# Autodesk Inventor assembly: robot
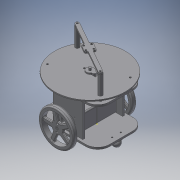
[picture p0: Inventor's stored thumbnail of the model, 180x180]
Saved by Autodesk Inventor 2017 (Build 210142000, 142)
## iProperties
Created: 2017-06-15
Part Number: robot
Document SubType Name: Assembly
Designer: millerid
Author: millerid
## Documents named in this file (13)
- U:\Research\Swarms\RobotModel\robot.iam
- U:\Research\Swarms\RobotModel\pcb.ipt
- U:\Research\Swarms\RobotModel\SG92R.ipt
- U:\Research\Swarms\RobotModel\NEMA11.ipt
- U:\Research\Swarms\RobotModel\halfincaster.ipt
- U:\Research\Swarms\RobotModel\1_5V_holder4AA.iam
- U:\Research\Swarms\RobotModel\Pololu 60mm Wheel.ipt
- U:\Research\Swarms\RobotModel\base_plate.ipt
- U:\Research\Swarms\RobotModel\side_plate.ipt
- U:\Research\Swarms\RobotModel\top_plate.ipt
- U:\Research\Swarms\RobotModel\quarterin_spacer.ipt
- U:\Research\Swarms\RobotModel\led_brace.ipt
- U:\Research\Swarms\RobotModel\oneandquarterstandoff.ipt
## Components (20 placed, 12 different names)
1. pcb:1 — Mate:46, Mate:47, Mate:48, Mate:64, Mate:65, Mate:67, Mate:70, Mate:71, Mate:72, Mate:73, Mate:74
2. SG92R:1 — Mate:46, Mate:47, Mate:70
3. NEMA11:1 — Mate:3, Mate:19
4. NEMA11:2 — Mate:14, Mate:15, Mate:20, Mate:61
5. halfincaster:1 — Mate:56, Mate:57
6. 1_5V_holder4AA:1 [sub-assembly] — Mate:60, Mate:61
7. Pololu 60mm Wheel:1 — Mate:3
8. halfincaster:2 — Mate:54, Mate:55, Mate:75
9. base_plate:1 — Mate:51, Mate:52, Mate:53, Mate:54, Mate:55, Mate:56, Mate:57, Mate:58, Mate:59, Mate:60, Mate:75
10. side_plate:1 — Mate:14, Mate:15, Mate:22, Mate:23, Mate:58, Mate:59
11. side_plate:2 — Mate:19
12. Pololu 60mm Wheel:2 — Mate:20
13. top_plate:1 — Mate:22, Mate:23, Mate:62, Mate:63, Mate:66, Mate:68, Mate:69
14. led_brace:1 — Mate:36, Mate:37, Mate:38, Mate:40
15. oneandquarterstandoff:1 — Mate:36, Mate:37, Mate:74
16. oneandquarterstandoff:2 — Mate:38, Mate:40, Mate:48, Mate:73
17. quarterin_spacer:1 — Mate:62, Mate:63, Mate:64, Mate:65
18. quarterin_spacer:2 — Mate:69, Mate:72
19. quarterin_spacer:3 — Mate:66, Mate:67
20. quarterin_spacer:4 — Mate:68, Mate:71
## Relationships (39: Mate 39)
- Mate:3: NEMA11:1 ↔ Pololu 60mm Wheel:1
- Mate:14: NEMA11:2 ↔ side_plate:1
- Mate:15: NEMA11:2 ↔ side_plate:1
- Mate:19: NEMA11:1 ↔ side_plate:2
- Mate:20: NEMA11:2 ↔ Pololu 60mm Wheel:2
- Mate:22: side_plate:1 ↔ top_plate:1
- Mate:23: side_plate:1 ↔ top_plate:1
- Mate:36: led_brace:1 ↔ oneandquarterstandoff:1
- Mate:37: led_brace:1 ↔ oneandquarterstandoff:1
- Mate:38 (0.1 mm): led_brace:1 ↔ oneandquarterstandoff:2
- Mate:40: led_brace:1 ↔ oneandquarterstandoff:2
- Mate:46: pcb:1 ↔ SG92R:1
- Mate:47: pcb:1 ↔ SG92R:1
- Mate:48: pcb:1 ↔ oneandquarterstandoff:2
- Mate:51: base_plate:1
- Mate:52: base_plate:1
- Mate:53: base_plate:1
- Mate:54: halfincaster:2 ↔ base_plate:1
- Mate:55: halfincaster:2 ↔ base_plate:1
- Mate:56: halfincaster:1 ↔ base_plate:1
- Mate:57: halfincaster:1 ↔ base_plate:1
- Mate:58: base_plate:1 ↔ side_plate:1
- Mate:59: base_plate:1 ↔ side_plate:1
- Mate:60: 1_5V_holder4AA:1 ↔ base_plate:1
- Mate:61: NEMA11:2 ↔ 1_5V_holder4AA:1
- Mate:62: top_plate:1 ↔ quarterin_spacer:1
- Mate:63: top_plate:1 ↔ quarterin_spacer:1
- Mate:64: pcb:1 ↔ quarterin_spacer:1
- Mate:65: pcb:1 ↔ quarterin_spacer:1
- Mate:66: top_plate:1 ↔ quarterin_spacer:3
- Mate:67: pcb:1 ↔ quarterin_spacer:3
- Mate:68: top_plate:1 ↔ quarterin_spacer:4
- Mate:69: top_plate:1 ↔ quarterin_spacer:2
- Mate:70 (0.2 mm): pcb:1 ↔ SG92R:1
- Mate:71: pcb:1 ↔ quarterin_spacer:4
- Mate:72: pcb:1 ↔ quarterin_spacer:2
- Mate:73: pcb:1 ↔ oneandquarterstandoff:2
- Mate:74: pcb:1 ↔ oneandquarterstandoff:1
- Mate:75: halfincaster:2 ↔ base_plate:1
